# Autodesk Inventor assembly: 조립품2
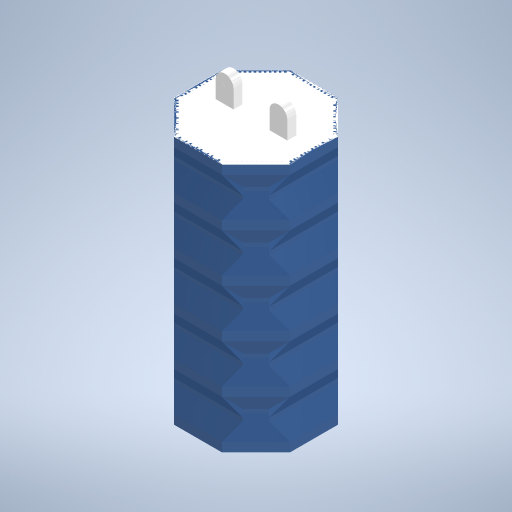
[picture p0: Inventor's stored thumbnail of the model, 512x512]
Saved by Autodesk Inventor 2024 (Build 280153000, 153)
## iProperties
Created: 2023-06-15
Part Number: 조립품2
Document SubType Name: Assembly
Designer: jsw
Author: jsw
## Documents named in this file (3)
- C:\승원\co-op\3rd_보근\Soft actuator\IPT,IAM\조립품2.iam
- C:\승원\co-op\3rd_보근\Soft actuator\IPT,IAM\ASSEMBLY_단순화_1.ipt
- C:\승원\co-op\3rd_보근\Soft actuator\IPT,IAM\부품10.ipt
## Components (2 placed, 2 different names)
1. ASSEMBLY_단순화_1:1 — 플러쉬:1, 플러쉬:2, 플러쉬:3, 플러쉬:4
2. 부품10:1 — 플러쉬:1, 플러쉬:2, 플러쉬:3, 플러쉬:4
## Relationships (4: Flush 4)
- 플러쉬:1 [Flush]: ASSEMBLY_단순화_1:1 ↔ 부품10:1
- 플러쉬:2 [Flush]: ASSEMBLY_단순화_1:1 ↔ 부품10:1
- 플러쉬:3 [Flush]: ASSEMBLY_단순화_1:1 ↔ 부품10:1
- 플러쉬:4 [Flush]: ASSEMBLY_단순화_1:1 ↔ 부품10:1
